# Autodesk Inventor assembly: VP-Input-775pro
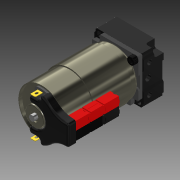
[picture p0: Inventor's stored thumbnail of the model, 180x180]
Saved by Autodesk Inventor 2022 (Build 260153000, 153)
## iProperties
Created: 2018-08-19
Part Number: VP-Input-775pro
Document SubType Name: Assembly
Mass: 418.235 g
Surface Area: 296.022 cm^2
Volume: 114.386 cm^3
Density: 3.65636 g/cm^3
## Documents named in this file (12)
- E:\Middleton Robotics\Collaborative Robots\Collaborative Part Library\General Gearboxes\Planetaries\Versaplanetary\V2 Stages\V2 Input Stage\VP 775pro Input.iam
- E:\Middleton Robotics\Collaborative Robots\Collaborative Part Library\General Gearboxes\Planetaries\Versaplanetary\V2 Stages\V2 Input Housing.ipt
- E:\Middleton Robotics\Collaborative Robots\Collaborative Part Library\General Gearboxes\Planetaries\Versaplanetary\Motor Mounting Plates\VP 775 Mounting Plate.ipt
- E:\Middleton Robotics\Collaborative Robots\Collaborative Part Library\General Gearboxes\Planetaries\Versaplanetary\Screws\M4 x 10mm Screw.ipt
- E:\Middleton Robotics\Collaborative Robots\Collaborative Part Library\Motors\FRC\775pro.ipt
- E:\Middleton Robotics\Collaborative Robots\Collaborative Part Library\General Gearboxes\Planetaries\Versaplanetary\Input Coupler\5mm Coupler Sleeve.ipt
- E:\Middleton Robotics\Collaborative Robots\Collaborative Part Library\General Gearboxes\Planetaries\Versaplanetary\Input Coupler\VP Input Coupler.ipt
- E:\Middleton Robotics\Collaborative Robots\Collaborative Part Library\General Gearboxes\Planetaries\Versaplanetary\Input Coupler\Coupler Set Screw.ipt
- E:\Middleton Robotics\Collaborative Robots\Collaborative Part Library\General Gearboxes\Planetaries\Versaplanetary\Screws\8-32 x 0.50in Screw.ipt
- E:\Middleton Robotics\Collaborative Robots\Collaborative Part Library\General Gearboxes\Planetaries\Versaplanetary\V2 Stages\V2 Input Stage\775_inline_connector_v1.ipt
- E:\Middleton Robotics\Collaborative Robots\Collaborative Part Library\General Gearboxes\Planetaries\Versaplanetary\V2 Stages\V2 Input Stage\PowerPoles.ipt
- E:\Middleton Robotics\Collaborative Robots\Collaborative Part Library\General Gearboxes\Planetaries\Versaplanetary\V2 Stages\V2 Input Stage.iam
## Components (12 placed, 10 different names)
1. V2 Input Housing:1 — Mate:1, Mate:2, Flush:1, Mate:13, Flush:5, Mate:14, Mate:15
2. VP 775 Mounting Plate:1 — Mate:1, Mate:2, Flush:1, Insert:1, Insert:2, Insert:5, Insert:6, Mate:17
3. M4 x 10mm Screw:1 — Insert:1
4. M4 x 10mm Screw:2 — Insert:2
5. 775pro:1 — Insert:5, Insert:6, Mate:20, Mate:21, Angle:3
6. 5mm Coupler Sleeve:1 — Insert:12, Angle:1
7. VP Input Coupler:1 — Angle:1, Mate:12, Tangent:1, Mate:13, Flush:5, Insert:12
8. Coupler Set Screw:1 — Mate:12, Tangent:1
9. 8-32 x 0.50in Screw:1 — Mate:14, Mate:17, Flush:6
10. 8-32 x 0.50in Screw:2 — Mate:15, Flush:6
11. 775_inline_connector_v1:1 — Mate:20, Mate:21, Angle:3, Mate:22, Flush:7, Flush:8
12. PowerPoles:1 — Mate:22, Flush:7, Flush:8
## Relationships (23: Mate 10, Flush 5, Insert 5, Angle 2, Tangent 1)
- Mate:1: V2 Input Housing:1 ↔ VP 775 Mounting Plate:1
- Mate:2: V2 Input Housing:1 ↔ VP 775 Mounting Plate:1
- Flush:1: V2 Input Housing:1 ↔ VP 775 Mounting Plate:1
- Insert:1: VP 775 Mounting Plate:1 ↔ M4 x 10mm Screw:1
- Insert:2: VP 775 Mounting Plate:1 ↔ M4 x 10mm Screw:2
- Insert:5: VP 775 Mounting Plate:1 ↔ 775pro:1
- Insert:6: VP 775 Mounting Plate:1 ↔ 775pro:1
- Insert:12: 5mm Coupler Sleeve:1 ↔ VP Input Coupler:1
- Angle:1 (0 deg): 5mm Coupler Sleeve:1 ↔ VP Input Coupler:1
- Mate:12: VP Input Coupler:1 ↔ Coupler Set Screw:1
- Tangent:1: VP Input Coupler:1 ↔ Coupler Set Screw:1
- Mate:13: V2 Input Housing:1 ↔ VP Input Coupler:1
- Flush:5 (2.4 mm): V2 Input Housing:1 ↔ VP Input Coupler:1
- Mate:14: V2 Input Housing:1 ↔ 8-32 x 0.50in Screw:1
- Mate:15: V2 Input Housing:1 ↔ 8-32 x 0.50in Screw:2
- Mate:17: VP 775 Mounting Plate:1 ↔ 8-32 x 0.50in Screw:1
- Flush:6: 8-32 x 0.50in Screw:1 ↔ 8-32 x 0.50in Screw:2
- Mate:20: 775pro:1 ↔ 775_inline_connector_v1:1
- Mate:21: 775pro:1 ↔ 775_inline_connector_v1:1
- Angle:3 (0 deg): 775pro:1 ↔ 775_inline_connector_v1:1
- Mate:22: 775_inline_connector_v1:1 ↔ PowerPoles:1
- Flush:7: 775_inline_connector_v1:1 ↔ PowerPoles:1
- Flush:8: 775_inline_connector_v1:1 ↔ PowerPoles:1
